# Autodesk Inventor assembly: all형상
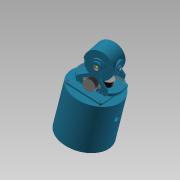
[picture p0: Inventor's stored thumbnail of the model, 180x180]
Saved by Autodesk Inventor 2018 (Build 220112000, 112)
## iProperties
Created: 2018-05-03
Part Number: all형상
Material: 일반
Document SubType Name: Assembly
Designer: CK
Author: CK
## Documents named in this file (3)
- C:\Users\CK\Desktop\캡스톤\all형상.iam
- C:\Users\CK\Desktop\캡스톤\상부조립.iam
- C:\Users\CK\Desktop\캡스톤\바텀조립.iam
## Components (2 placed, 2 different names)
1. 상부조립:1 [sub-assembly] — 메이트:1, 메이트:2, 메이트:3
2. 바텀조립:1 [sub-assembly] — 메이트:1, 메이트:2, 메이트:3
## Relationships (3: Mate 3)
- 메이트:1 [Mate]: 상부조립:1 ↔ 바텀조립:1
- 메이트:2 [Mate]: 상부조립:1 ↔ 바텀조립:1
- 메이트:3 [Mate]: 상부조립:1 ↔ 바텀조립:1
